# Autodesk Inventor assembly: Configuration 1
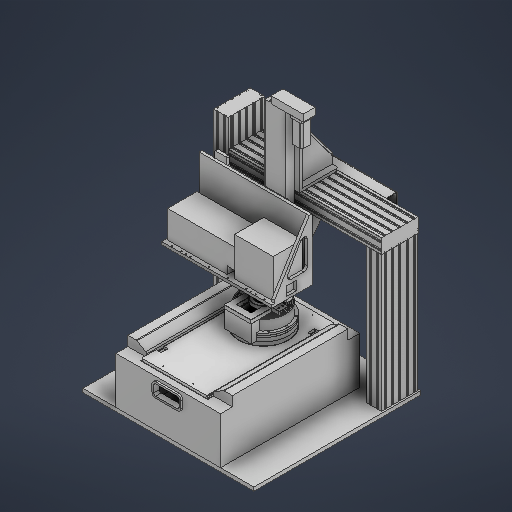
[picture p0: Inventor's stored thumbnail of the model, 512x512]
Saved by Autodesk Inventor 2025 (Build 290162000, 162)
## iProperties
Created: 2024-06-05
Part Number: Configuration 1
Document SubType Name: Assembly
Designer: AdminForWorker
Title: Printer Assembly v13
Author: AdminForWorker
## Documents named in this file (30)
- C:\Users\mayhe\OneDrive\Documents\GitHub\In-situ-monitoring-of-powder-bed-fusion-additive-manufacturing\system_development\Orichalcum\v0.2\Hardware_design\Full Printer Assembly\Printer Assembly.iam
- C:\Users\mayhe\OneDrive\Documents\GitHub\In-situ-monitoring-of-powder-bed-fusion-additive-manufacturing\system_development\Orichalcum\v0.2\Hardware_design\Full Printer Assembly\Printer Body v6.ipt
- C:\Users\mayhe\OneDrive\Documents\GitHub\In-situ-monitoring-of-powder-bed-fusion-additive-manufacturing\system_development\Orichalcum\v0.2\Hardware_design\Full Printer Assembly\Printer Frame.ipt
- C:\Users\mayhe\OneDrive\Documents\GitHub\In-situ-monitoring-of-powder-bed-fusion-additive-manufacturing\system_development\Orichalcum\v0.2\Hardware_design\Full Printer Assembly\overhead laser unit v1.ipt
- C:\Users\mayhe\OneDrive\Documents\GitHub\In-situ-monitoring-of-powder-bed-fusion-additive-manufacturing\system_development\Orichalcum\v0.2\Hardware_design\Full Printer Assembly\Part4.ipt
- C:\Users\mayhe\OneDrive\Documents\GitHub\In-situ-monitoring-of-powder-bed-fusion-additive-manufacturing\system_development\Orichalcum\v0.2\Hardware_design\custom-cover\cover\Updated Cover.ipt
- C:\Users\mayhe\OneDrive\Documents\GitHub\In-situ-monitoring-of-powder-bed-fusion-additive-manufacturing\system_development\Orichalcum\v0.2\Hardware_design\custom-cover\cylinder-parts\final-parts\Cylinder Bottom Ring.ipt
- C:\Users\mayhe\OneDrive\Documents\GitHub\In-situ-monitoring-of-powder-bed-fusion-additive-manufacturing\system_development\Orichalcum\v0.2\Hardware_design\custom-cover\cylinder-parts\final-parts\Cylinder Spacer 25mm.ipt
- C:\Users\mayhe\OneDrive\Documents\GitHub\In-situ-monitoring-of-powder-bed-fusion-additive-manufacturing\system_development\Orichalcum\v0.2\Hardware_design\custom-cover\cylinder-parts\final-parts\Cylinder Slidey Bit Housing.ipt
- C:\Users\mayhe\OneDrive\Documents\GitHub\In-situ-monitoring-of-powder-bed-fusion-additive-manufacturing\system_development\Orichalcum\v0.2\Hardware_design\custom-cover\cylinder-parts\cylinder-segments\Cylinder Segment - 01.ipt
- C:\Users\mayhe\OneDrive\Documents\GitHub\In-situ-monitoring-of-powder-bed-fusion-additive-manufacturing\system_development\Orichalcum\v0.2\Hardware_design\custom-cover\cylinder-parts\cylinder-segments\Cylinder Segment .ipt
- C:\Users\mayhe\OneDrive\Documents\GitHub\In-situ-monitoring-of-powder-bed-fusion-additive-manufacturing\system_development\Orichalcum\v0.2\Hardware_design\custom-cover\cylinder-parts\cylinder-segments\Cylinder Segment - 02.ipt
- C:\Users\mayhe\OneDrive\Documents\GitHub\In-situ-monitoring-of-powder-bed-fusion-additive-manufacturing\system_development\Orichalcum\v0.2\Hardware_design\custom-cover\cylinder-parts\cylinder-segments\Cylinder Segment - 03.ipt
- C:\Users\mayhe\OneDrive\Documents\GitHub\In-situ-monitoring-of-powder-bed-fusion-additive-manufacturing\system_development\Orichalcum\v0.2\Hardware_design\custom-cover\cylinder-parts\cylinder-segments\Cylinder Segment - 04.ipt
- C:\Users\mayhe\OneDrive\Documents\GitHub\In-situ-monitoring-of-powder-bed-fusion-additive-manufacturing\system_development\Orichalcum\v0.2\Hardware_design\custom-cover\cylinder-parts\cylinder-segments\Cylinder Segment - 05.ipt
- C:\Users\mayhe\OneDrive\Documents\GitHub\In-situ-monitoring-of-powder-bed-fusion-additive-manufacturing\system_development\Orichalcum\v0.2\Hardware_design\custom-cover\cylinder-parts\cylinder-segments\Cylinder Segment - 06.ipt
- C:\Users\mayhe\OneDrive\Documents\GitHub\In-situ-monitoring-of-powder-bed-fusion-additive-manufacturing\system_development\Orichalcum\v0.2\Hardware_design\custom-cover\cylinder-parts\cylinder-segments\Cylinder Segment - 07.ipt
- C:\Users\mayhe\OneDrive\Documents\GitHub\In-situ-monitoring-of-powder-bed-fusion-additive-manufacturing\system_development\Orichalcum\v0.2\Hardware_design\custom-cover\cylinder-parts\cylinder-segments\Cylinder Segment - 08.ipt
- C:\Users\mayhe\OneDrive\Documents\GitHub\In-situ-monitoring-of-powder-bed-fusion-additive-manufacturing\system_development\Orichalcum\v0.2\Hardware_design\custom-cover\cylinder-parts\cylinder-segments\Cylinder Segment - 09.ipt
- C:\Users\mayhe\OneDrive\Documents\GitHub\In-situ-monitoring-of-powder-bed-fusion-additive-manufacturing\system_development\Orichalcum\v0.2\Hardware_design\custom-cover\cylinder-parts\cylinder-segments\Cylinder Segment - 10.ipt
- C:\Users\mayhe\OneDrive\Documents\GitHub\In-situ-monitoring-of-powder-bed-fusion-additive-manufacturing\system_development\Orichalcum\v0.2\Hardware_design\custom-cover\cylinder-parts\cylinder-segments\Cylinder Segment - Face.ipt
- C:\Users\mayhe\OneDrive\Documents\GitHub\In-situ-monitoring-of-powder-bed-fusion-additive-manufacturing\system_development\Orichalcum\v0.2\Hardware_design\custom-cover\cylinder-parts\Galvo Housing\Galvo Housing 4\Galvo Housing-01.ipt
- C:\Users\mayhe\OneDrive\Documents\GitHub\In-situ-monitoring-of-powder-bed-fusion-additive-manufacturing\system_development\Orichalcum\v0.2\Hardware_design\custom-cover\cylinder-parts\Galvo Housing\Galvo Housing 4.ipt
- C:\Users\mayhe\OneDrive\Documents\GitHub\In-situ-monitoring-of-powder-bed-fusion-additive-manufacturing\system_development\Orichalcum\v0.2\Hardware_design\custom-cover\cylinder-parts\Galvo Housing\Galvo Housing 1\Galvo Housing-01.ipt
- C:\Users\mayhe\OneDrive\Documents\GitHub\In-situ-monitoring-of-powder-bed-fusion-additive-manufacturing\system_development\Orichalcum\v0.2\Hardware_design\custom-cover\cylinder-parts\Galvo Housing\Galvo Housing 1.ipt
- C:\Users\mayhe\OneDrive\Documents\GitHub\In-situ-monitoring-of-powder-bed-fusion-additive-manufacturing\system_development\Orichalcum\v0.2\Hardware_design\custom-cover\cylinder-parts\Galvo Housing\Galvo Housing 2\Galvo Housing-01.ipt
- C:\Users\mayhe\OneDrive\Documents\GitHub\In-situ-monitoring-of-powder-bed-fusion-additive-manufacturing\system_development\Orichalcum\v0.2\Hardware_design\custom-cover\cylinder-parts\Galvo Housing\Galvo Housing 2.ipt
- C:\Users\mayhe\OneDrive\Documents\GitHub\In-situ-monitoring-of-powder-bed-fusion-additive-manufacturing\system_development\Orichalcum\v0.2\Hardware_design\custom-cover\cylinder-parts\Galvo Housing\Galvo Housing 3\Galvo Housing-01.ipt
- C:\Users\mayhe\OneDrive\Documents\GitHub\In-situ-monitoring-of-powder-bed-fusion-additive-manufacturing\system_development\Orichalcum\v0.2\Hardware_design\custom-cover\cylinder-parts\Galvo Housing\Galvo Housing 3.ipt
- C:\Users\mayhe\OneDrive\Documents\GitHub\In-situ-monitoring-of-powder-bed-fusion-additive-manufacturing\system_development\Orichalcum\v0.2\Hardware_design\custom-cover\cylinder-parts\Galvo Housing\Spacer 1.ipt
## Components (24 placed, 21 different names)
1. Printer Frame:1 — Flush:1, Mate:1, Mate:2, Mate:3, Flush:2, Flush:3
2. Printer Body v6:1 — Flush:1, Mate:1, Mate:2, Mate:5, Mate:6, Mate:7, Angle:12
3. overhead laser unit v1:1 — Mate:4, Angle:1, Flush:4
4. Part4:1 — Mate:3, Flush:2, Flush:3, Mate:4, Angle:1, Flush:4
5. Updated Cover:1 — Mate:5, Mate:6, Mate:7, Rotational:1, Mate:8
6. Cylinder Bottom Ring:1 — Rotational:1, Mate:8, Rotational:2, Mate:9, Mate:22
7. Cylinder Spacer 25mm:1 — Rotational:2, Mate:9, Rotational:3, Mate:10
8. Cylinder Slidey Bit Housing:1 — Rotational:4, Mate:21, Mate:23
9. Cylinder Segment - 01:1 — Rotational:3, Mate:10, Mate:11, Angle:2, Rotational:4, Mate:21
10. Cylinder Segment - 02:2 — Mate:11, Mate:12, Angle:2, Angle:3
11. Cylinder Segment - 03:3 — Mate:12, Mate:13, Angle:3, Angle:4, Angle:6, Angle:7
12. Cylinder Segment - 04:4 — Mate:13, Mate:14, Angle:4, Angle:5
13. Cylinder Segment - 05:5 — Mate:14, Mate:15, Angle:5
14. Cylinder Segment - 06:6 — Mate:15, Mate:16, Angle:6
15. Cylinder Segment - 07:7 — Mate:16, Mate:17, Angle:7, Angle:8
16. Cylinder Segment - 08:8 — Mate:17, Mate:18, Angle:8, Angle:9, Mate:24
17. Cylinder Segment - 09:9 — Mate:18, Mate:19, Angle:9, Angle:10, Mate:27
18. Cylinder Segment - 10:10 — Mate:19, Mate:20, Angle:10, Angle:11
19. Cylinder Segment - Face:11 — Mate:20, Angle:11, Mate:25, Mate:29
20. Galvo Housing-01:1 — Mate:22, Mate:23, Mate:24, Mate:26
21. Galvo Housing-01:1 — Mate:25, Mate:26, Mate:28
22. Galvo Housing-01:1 — Mate:27, Mate:28, Mate:30
23. Galvo Housing-01:1 — Mate:29, Mate:30, Rotational:5
24. Spacer 1:1 — Rotational:5, Angle:12
## Relationships (51: Mate 30, Angle 12, RevoluteJoint 5, Flush 4)
- Flush:1: Printer Frame:1 ↔ Printer Body v6:1
- Mate:1: Printer Frame:1 ↔ Printer Body v6:1
- Mate:2 (92.5 mm): Printer Frame:1 ↔ Printer Body v6:1
- Mate:3: Printer Frame:1 ↔ Part4:1
- Flush:2 (28.5 mm): Printer Frame:1 ↔ Part4:1
- Flush:3 (-27 mm): Printer Frame:1 ↔ Part4:1
- Mate:4: overhead laser unit v1:1 ↔ Part4:1
- Angle:1 (179.9998 deg): overhead laser unit v1:1 ↔ Part4:1
- Flush:4 (-30 mm): overhead laser unit v1:1 ↔ Part4:1
- Mate:5: Printer Body v6:1 ↔ Updated Cover:1
- Mate:6: Printer Body v6:1 ↔ Updated Cover:1
- Mate:7: Printer Body v6:1 ↔ Updated Cover:1
- Rotational:1 [RevoluteJoint]: Updated Cover:1 ↔ Cylinder Bottom Ring:1
- Mate:8: Updated Cover:1 ↔ Cylinder Bottom Ring:1
- Rotational:2 [RevoluteJoint]: Cylinder Bottom Ring:1 ↔ Cylinder Spacer 25mm:1
- Mate:9: Cylinder Bottom Ring:1 ↔ Cylinder Spacer 25mm:1
- Rotational:3 [RevoluteJoint]: Cylinder Spacer 25mm:1 ↔ Cylinder Segment - 01:1
- Mate:10: Cylinder Spacer 25mm:1 ↔ Cylinder Segment - 01:1
- Mate:11: Cylinder Segment - 01:1 ↔ Cylinder Segment - 02:2
- Mate:12: Cylinder Segment - 02:2 ↔ Cylinder Segment - 03:3
- Mate:13: Cylinder Segment - 03:3 ↔ Cylinder Segment - 04:4
- Mate:14: Cylinder Segment - 04:4 ↔ Cylinder Segment - 05:5
- Mate:15: Cylinder Segment - 05:5 ↔ Cylinder Segment - 06:6
- Mate:16: Cylinder Segment - 06:6 ↔ Cylinder Segment - 07:7
- Mate:17: Cylinder Segment - 07:7 ↔ Cylinder Segment - 08:8
- Mate:18: Cylinder Segment - 08:8 ↔ Cylinder Segment - 09:9
- Mate:19: Cylinder Segment - 09:9 ↔ Cylinder Segment - 10:10
- Mate:20: Cylinder Segment - 10:10 ↔ Cylinder Segment - Face:11
- Angle:2 (0 deg): Cylinder Segment - 01:1 ↔ Cylinder Segment - 02:2
- Angle:3 (0 deg): Cylinder Segment - 02:2 ↔ Cylinder Segment - 03:3
- Angle:4 (0 deg): Cylinder Segment - 03:3 ↔ Cylinder Segment - 04:4
- Angle:5 (0 deg): Cylinder Segment - 04:4 ↔ Cylinder Segment - 05:5
- Angle:6 (0 deg): Cylinder Segment - 03:3 ↔ Cylinder Segment - 06:6
- Angle:7 (0 deg): Cylinder Segment - 03:3 ↔ Cylinder Segment - 07:7
- Angle:8 (0 deg): Cylinder Segment - 07:7 ↔ Cylinder Segment - 08:8
- Angle:9 (0 deg): Cylinder Segment - 08:8 ↔ Cylinder Segment - 09:9
- Angle:10 (0 deg): Cylinder Segment - 09:9 ↔ Cylinder Segment - 10:10
- Angle:11 (0 deg): Cylinder Segment - 10:10 ↔ Cylinder Segment - Face:11
- Rotational:4 [RevoluteJoint]: Cylinder Slidey Bit Housing:1 ↔ Cylinder Segment - 01:1
- Mate:21: Cylinder Slidey Bit Housing:1 ↔ Cylinder Segment - 01:1
- Mate:22: Cylinder Bottom Ring:1 ↔ Galvo Housing-01:1
- Mate:23: Cylinder Slidey Bit Housing:1 ↔ Galvo Housing-01:1
- Mate:24: Cylinder Segment - 08:8 ↔ Galvo Housing-01:1
- Mate:25 (0.5 mm): Cylinder Segment - Face:11 ↔ Galvo Housing-01:1
- Mate:26 (0.5 mm): Galvo Housing-01:1
- Mate:27 (0.5 mm): Cylinder Segment - 09:9 ↔ Galvo Housing-01:1
- Mate:28 (0.5 mm): Galvo Housing-01:1
- Mate:29 (0.5 mm): Cylinder Segment - Face:11 ↔ Galvo Housing-01:1
- Mate:30 (0.5 mm): Galvo Housing-01:1
- Rotational:5 [RevoluteJoint]: Galvo Housing-01:1 ↔ Spacer 1:1
- Angle:12 (0 deg): Printer Body v6:1 ↔ Spacer 1:1
